# Autodesk Inventor assembly: Arm_Link_8
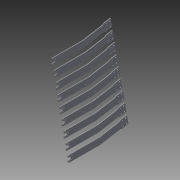
[picture p0: Inventor's stored thumbnail of the model, 180x180]
Saved by Autodesk Inventor 2013 (Build 170138000, 138)
## iProperties
Created: 2014-05-18
Part Number: Arm_Link_8
Document SubType Name: Assembly
Designer: andou
Author: andou
## Documents named in this file (2)
- C:\Users\andou\Documents\Inventor\RoboticsProject\project_4\Robot\Arm\Arm_Link_8.iam
- C:\Users\andou\Documents\Inventor\RoboticsProject\project_4\Robot\Arm\Arm_Link.ipt
## Components (9 placed, 1 different names)
1. Arm_Link:1
2. Arm_Link:2
3. Arm_Link:3
4. Arm_Link:4
5. Arm_Link:5
6. Arm_Link:6
7. Arm_Link:7
8. Arm_Link:8
9. Arm_Link:9
## Component patterns: (9 elements, first: Arm_Link:1)
